# Autodesk Inventor assembly: Hand_tyokudou
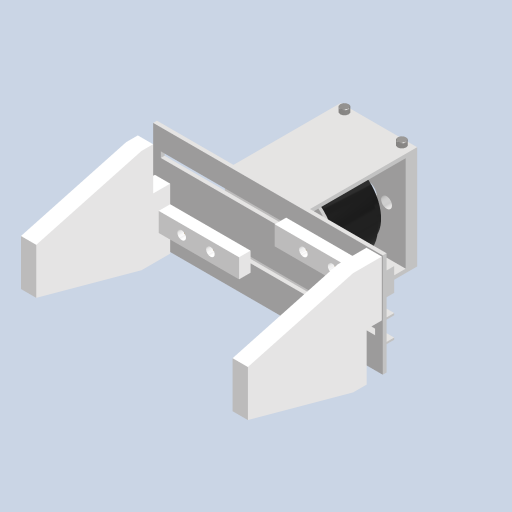
[picture p0: Inventor's stored thumbnail of the model, 512x512]
Saved by Autodesk Inventor 2023 (Build 270158000, 158)
## iProperties
Created: 2024-11-27
Part Number: Hand_tyokudou
Document SubType Name: Assembly
Designer: kiyo
Author: kiyo
## Documents named in this file (13)
- D:\GitHub\inventor\syu-si\OfficeRobot\Manipulator\Hand_tyokudou.iam
- D:\GitHub\inventor\syu-si\OfficeRobot\ReadyMade\Steadywin\GIM3505-8_with-driver.ipt
- D:\GitHub\inventor\syu-si\OfficeRobot\Manipulator\rackgear.ipt
- D:\GitHub\inventor\syu-si\OfficeRobot\Manipulator\motor-fixing.ipt
- D:\GitHub\inventor\syu-si\OfficeRobot\Manipulator\hand-box.ipt
- D:\GitHub\inventor\syu-si\OfficeRobot\Manipulator\left-nail.ipt
- D:\GitHub\inventor\syu-si\OfficeRobot\Manipulator\right-nail.ipt
- D:\GitHub\inventor\syu-si\OfficeRobot\Manipulator\hand-gear.ipt
- D:\GitHub\inventor\syu-si\OfficeRobot\ReadyMade\Screw\GFM-0304-03.ipt
- D:\GitHub\inventor\syu-si\OfficeRobot\ReadyMade\Screw\FB-305530.ipt
- D:\GitHub\inventor\syu-si\OfficeRobot\ReadyMade\Screw\CBSH3-8.ipt
- D:\GitHub\inventor\syu-si\OfficeRobot\ReadyMade\Screw\M2-5_6mm.ipt
- D:\GitHub\inventor\syu-si\OfficeRobot\Manipulator\connect-wrist.ipt
## Components (33 placed, 12 different names)
1. GIM3505-8_with-driver:1 — 角度:3, 挿入:2, 挿入:3
2. left-nail:1 — 挿入:10, 挿入:11, 挿入:20, 挿入:21
3. right-nail:1 — 挿入:14, 挿入:15, 挿入:18, 挿入:19
4. hand-box:1 — メイト:8, メイト:9, 挿入:28, 挿入:29, 挿入:34, 挿入:35, 挿入:36, 挿入:37, 挿入:38, 挿入:39
5. rackgear:1 — 角度:2, 挿入:16, 挿入:17, 挿入:24, 挿入:25
6. rackgear:2 — 角度:1, 挿入:12, 挿入:13, 挿入:22, 挿入:23
7. hand-gear
8. motor-fixing:1 — 挿入:2, 挿入:3, 挿入:26, 挿入:27
9. GFM-0304-03:1 — 挿入:10, 挿入:13, メイト:8
10. GFM-0304-03:2 — 挿入:11, 挿入:12
11. GFM-0304-03:3 — 挿入:14, メイト:9, 挿入:16
12. GFM-0304-03:4 — 挿入:15, 挿入:17
13. FB-305530:1 — 挿入:18
14. FB-305530:2 — 挿入:19
15. FB-305530:3 — 挿入:21
16. FB-305530:4 — 挿入:20
17. CBSH3-8:1 — 挿入:25
18. CBSH3-8:2 — 挿入:24
19. CBSH3-8:3 — 挿入:23
20. CBSH3-8:4 — 挿入:22
21. FB-305530:5 — 挿入:27
22. FB-305530:6 — 挿入:26
23. M2-5_6mm:1 — 挿入:28
24. M2-5_6mm:2 — 挿入:29
25. connect-wrist:1 — 挿入:30, 挿入:31, 挿入:32, 挿入:33, 挿入:34
26. FB-305530:7 — 挿入:31
27. FB-305530:8 — 挿入:30, 挿入:35
28. FB-305530:9 — 挿入:33
29. FB-305530:10 — 挿入:32
30. M2-5_6mm:3 — 挿入:37
31. M2-5_6mm:4 — 挿入:36
32. M2-5_6mm:5 — 挿入:39
33. M2-5_6mm:6 — 挿入:38
## Relationships (42: Insert 35, Mate 4, Angle 3)
- 角度:1 [Angle] (0 deg): rackgear:2
- 角度:2 [Angle] (180 deg): rackgear:1
- [Insert]: GIM3505-8_with-driver:1 ↔ hand-gear
- [Mate] (0.05 mm): hand-box:1 ↔ rackgear:2
- [Mate] (0.05 mm): hand-box:1 ↔ rackgear:1
- 角度:3 [Angle] (0 deg): GIM3505-8_with-driver:1
- 挿入:2 [Insert]: GIM3505-8_with-driver:1 ↔ motor-fixing:1
- 挿入:3 [Insert]: GIM3505-8_with-driver:1 ↔ motor-fixing:1
- [Insert]: hand-box:1 ↔ motor-fixing:1
- [Insert]: hand-box:1 ↔ motor-fixing:1
- 挿入:10 [Insert]: left-nail:1 ↔ GFM-0304-03:1
- 挿入:11 [Insert]: left-nail:1 ↔ GFM-0304-03:2
- 挿入:12 [Insert]: rackgear:2 ↔ GFM-0304-03:2
- 挿入:13 [Insert]: rackgear:2 ↔ GFM-0304-03:1
- メイト:8 [Mate]: hand-box:1 ↔ GFM-0304-03:1
- 挿入:14 [Insert]: right-nail:1 ↔ GFM-0304-03:3
- 挿入:15 [Insert]: right-nail:1 ↔ GFM-0304-03:4
- メイト:9 [Mate]: hand-box:1 ↔ GFM-0304-03:3
- 挿入:16 [Insert]: rackgear:1 ↔ GFM-0304-03:3
- 挿入:17 [Insert]: rackgear:1 ↔ GFM-0304-03:4
- 挿入:18 [Insert]: right-nail:1 ↔ FB-305530:1
- 挿入:19 [Insert]: right-nail:1 ↔ FB-305530:2
- 挿入:20 [Insert]: left-nail:1 ↔ FB-305530:4
- 挿入:21 [Insert]: left-nail:1 ↔ FB-305530:3
- 挿入:22 [Insert]: rackgear:2 ↔ CBSH3-8:4
- 挿入:23 [Insert]: rackgear:2 ↔ CBSH3-8:3
- 挿入:24 [Insert]: rackgear:1 ↔ CBSH3-8:2
- 挿入:25 [Insert]: rackgear:1 ↔ CBSH3-8:1
- 挿入:26 [Insert]: motor-fixing:1 ↔ FB-305530:6
- 挿入:27 [Insert]: motor-fixing:1 ↔ FB-305530:5
- 挿入:28 [Insert]: hand-box:1 ↔ M2-5_6mm:1
- 挿入:29 [Insert]: hand-box:1 ↔ M2-5_6mm:2
- 挿入:30 [Insert]: connect-wrist:1 ↔ FB-305530:8
- 挿入:31 [Insert]: connect-wrist:1 ↔ FB-305530:7
- 挿入:32 [Insert]: connect-wrist:1 ↔ FB-305530:10
- 挿入:33 [Insert]: connect-wrist:1 ↔ FB-305530:9
- 挿入:34 [Insert]: hand-box:1 ↔ connect-wrist:1
- 挿入:35 [Insert]: hand-box:1 ↔ FB-305530:8
- 挿入:36 [Insert]: hand-box:1 ↔ M2-5_6mm:4
- 挿入:37 [Insert]: hand-box:1 ↔ M2-5_6mm:3
- 挿入:38 [Insert]: hand-box:1 ↔ M2-5_6mm:6
- 挿入:39 [Insert]: hand-box:1 ↔ M2-5_6mm:5
